# Autodesk Inventor assembly: dome_assembly
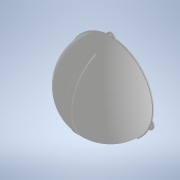
[picture p0: Inventor's stored thumbnail of the model, 180x180]
Saved by Autodesk Inventor 2021 (Build 250183000, 183)
## iProperties
Created: 2021-02-02
Part Number: dome_assembly
Document SubType Name: Assembly
Designer: dsdan
Author: dsdan
## Documents named in this file (3)
- E:\OneDrive - Imperial College London\DragonVision_DanielKo\Instrumentation\Ephys_rig_2021\dome_assembly.iam
- E:\OneDrive - Imperial College London\DragonVision_DanielKo\Instrumentation\Ephys_rig_2021\dome_mirror.ipt
- E:\OneDrive - Imperial College London\DragonVision_DanielKo\Instrumentation\Ephys_rig_2021\dome.ipt
## Components (2 placed, 2 different names)
1. dome_mirror:1 — Mate:1, Mate:2, Flush:1
2. dome:1 — Mate:1, Mate:2, Flush:1
## Relationships (3: Mate 2, Flush 1)
- Mate:1: dome_mirror:1 ↔ dome:1
- Mate:2: dome_mirror:1 ↔ dome:1
- Flush:1: dome_mirror:1 ↔ dome:1
